# Autodesk Inventor assembly: SCST8-8
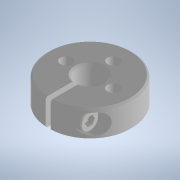
[picture p0: Inventor's stored thumbnail of the model, 180x180]
Saved by Autodesk Inventor 2021 (Build 250183000, 183)
## iProperties
Category: PARTsolutions
Company: MISUMI
Created: 2025-09-06
Part Number: SCST8-8
Catalog Web Link: www.cadenas.de
Description: SCST, PSCST, SSCST, SCSTR, PSCSTR, SSCSTR-Set Collars - Slit 3 Hole/3 Tap - Standard Type -
Vendor: MISUMI
Document SubType Name: Assembly
Designer: psAdmin
Manufacturer: MISUMI
Mass: 3.10789 g
Surface Area: 23.1514 cm^2
Volume: 3.10789 cm^3
Density: 1 g/cm^3
Title: SCST8-8
Author: Cadenas PARTsolutions
Comments: Set Collars - Slit 3 Hole/3 Tap - Standard Type -
PSOL_IDENT_0: {$CADENAS_DATA/23d-libs/misumi/metric/03_set_collars/scst_asmtab.prj},217 {VTYP=3D},{STYP=ASSTAB},{N
PSOL_IDENT_1: B=SCST8-8},{LINA=SCST8-8},{NN=SCST, PSCST, SSCST, SCSTR, PSCSTR, SSCSTR},{DATE=29.11.2024 04:05:21},
PSOL_IDENT_2: {GEOMDATE=15.09.2021 06:07:55},{VERSION=},{LINEID=50},{WBVAR=TS,MAT,ST,BS},{WBNUMERIC=BS}  {NB=SCST8
PSOL_IDENT_3: -8},{LINA=SCST8-8},{KT=DUMMY},{PN=SCST8-8},{TYPE=SCST},{TS=3H},{TSALG= '3H' , '3-Hole' , '3T' , '3-T
PSOL_IDENT_4: apped' },{MAT=S45C},{ST=BO},{STALG= 'BO' , 'Black Oxide' , 'ENP' , 'Electroless Nickel Plating' },{A
PSOL_IDENT_5: C=Hex Socket Head Cap Screw 1 pc.},{ACMAT=4137 Alloy Steel},{D=8},{BS=8},{BALG= 8 , 10 , 15 },{D1=25
PSOL_IDENT_6: },{M=M3},{M3D=3},{DD=3.4},{R=3.00},{W=1.5},{X=8.0},{Y=5},{P=14},{C=0.5},{S=3.5},{M1=-},{M13D=0},{L=1
PSOL_IDENT_7: 2},{PPATH=scst/scst_templ.prj}
NB: SCST8-8
NN: SCST, PSCST, SSCST, SCSTR, PSCSTR, SSCSTR
NT: Set Collars - Slit 3 Hole/3 Tap - Standard Type -
NBSYN: $PN.
LINA: SCST8-8
CATALOG: Misumi
PN: SCST8-8
TS: 3-Hole
MAT: 1045 Carbon Steel
ST: Black Oxide
AC: Hex Socket Head Cap Screw 1 pc.
ACMAT: 4137 Alloy Steel
D: 8
BS: 8
D1: 25
M: M3
DD: 3.4
R: 3
W: 1.5
X: 8
Y: 5
P: 14
C: 0.5
S: 3.5
M1: -
SUPPLIER: MISUMI
ARTICLENO: SCST8-8
BOMINFO: SCST8-8
CREATOR: CADENAS GmbH
## Documents named in this file (3)
- e:\temp\worker_COMMON_115\temp\tmp_9156_280_unfdc\format_0\SCST8-8.iam
- e:\temp\worker_COMMON_115\temp\tmp_9156_280_unfdc\format_0\SCST8-8b.ipt
- e:\temp\worker_COMMON_115\temp\tmp_9156_280_unfdc\format_0\BOLT3-12.ipt
## Components (2 placed, 2 different names)
1. SCST8-8b:1 — to_bolt_XY@1 <-> to_cp_XY@2, to_bolt_Z@1 <-> to_cp_Z@2, to_bolt_YZ@1 <-> to_cp_YZ@2
2. BOLT3-12:1 — to_bolt_XY@1 <-> to_cp_XY@2, to_bolt_Z@1 <-> to_cp_Z@2, to_bolt_YZ@1 <-> to_cp_YZ@2
## Relationships (3: Mate 2, Angle 1)
- to_bolt_XY@1 <-> to_cp_XY@2 [Mate]: SCST8-8b:1 ↔ BOLT3-12:1
- to_bolt_Z@1 <-> to_cp_Z@2 [Mate]: SCST8-8b:1 ↔ BOLT3-12:1
- to_bolt_YZ@1 <-> to_cp_YZ@2 [Angle] (0 deg): SCST8-8b:1 ↔ BOLT3-12:1
